# Autodesk Inventor assembly: Clamp with Piston Assembly arpan style
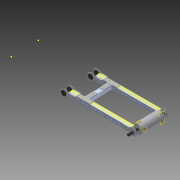
[picture p0: Inventor's stored thumbnail of the model, 180x180]
Saved by Autodesk Inventor 2014 SP1 (Build 180222100, 222)
## iProperties
Created: 2014-01-12
Part Number: Clamp with Piston Assembly arpan style
Document SubType Name: Assembly
Designer: Michael
Mass: 675.185 g
Surface Area: 3066.09 cm^2
Volume: 214.677 cm^3
Density: 3.14511 g/cm^3
Author: Michael
## Documents named in this file (12)
- C:\Users\Arpan\Documents\GitHub\2014buildCAD\New Collector\Clamp with Piston Assembly arpan style.iam
- C:\Users\Arpan\Documents\GitHub\2014buildCAD\New Collector\Vex Pro 1x1 rectangular tubing 14 in length.ipt
- C:\Users\Arpan\Documents\GitHub\2014buildCAD\New Collector\Vex Pro End Bearing Mount.ipt
- C:\Users\Arpan\Documents\GitHub\2014buildCAD\New Collector\Bearing Mount Spacer 1-8 in.ipt
- C:\Users\Arpan\Documents\GitHub\2014buildCAD\New Collector\Vex Pro 1x1 rectangular tubing 6 in length.ipt
- C:\Users\Arpan\Documents\GitHub\2014buildCAD\New Collector\Hex Bearing 3-8 in (FR6ZZL-hex (am-0692)).ipt
- C:\Users\Arpan\Documents\GitHub\2014buildCAD\New Shooter\Vex Pro T gusset.ipt
- C:\Users\Arpan\Documents\GitHub\2014buildCAD\New Shooter\Vex Pro End Bearing Mount.ipt
- C:\Users\Arpan\Documents\GitHub\2014buildCAD\New Shooter\Bearing ID 0.500 Hex OD 1.125.ipt
- C:\Users\Arpan\Documents\GitHub\2014buildCAD\sling shooter\Hex Shaft 1-2 in (am-0856).ipt
- C:\Users\Arpan\Documents\GitHub\2014buildCAD\sling shooter\roller.ipt
- C:\Users\Arpan\Documents\GitHub\2014buildCAD\sling shooter\insert.ipt
## Components (31 placed, 10 different names)
1. Vex Pro 1x1 rectangular tubing 14 in length:1 — Mate:128, Mate:129, Mate:130, Mate:131, Mate:132, Mate:133, Flush:1, Mate:173, Mate:174, Mate:176, Mate:177, Mate:180, Flush:4, Mate:186, Mate:190, Mate:191
2. Vex Pro 1x1 rectangular tubing 14 in length:2 — Mate:150, Mate:151, Mate:152, Mate:153, Mate:154, Mate:155, Mate:172, Flush:2, Flush:3, Mate:182, Mate:187, Mate:188, Mate:189, Mate:196, Mate:197, Mate:205
3. Vex Pro End Bearing Mount:3 — Mate:88, Mate:89, Mate:90, Mate:162, Mate:163
4. Vex Pro End Bearing Mount:4 — Mate:85, Mate:86, Mate:87, Mate:160, Mate:161
5. Bearing Mount Spacer 1-8 in:1 — Mate:85, Mate:86, Mate:87, Mate:125, Mate:126, Mate:127
6. Bearing Mount Spacer 1-8 in:2 — Mate:88, Mate:89, Mate:90, Mate:122, Mate:123, Mate:124
7. Vex Pro 1x1 rectangular tubing 6 in length:2 — Flush:1, Mate:172, Mate:173, Mate:175, Mate:178, Flush:3, Mate:179, Mate:181, Mate:198
8. Bearing Mount Spacer 1-8 in:5 — Mate:122, Mate:123, Mate:124, Mate:128, Mate:129, Mate:130
9. Bearing Mount Spacer 1-8 in:6 — Mate:125, Mate:126, Mate:127, Mate:131, Mate:132, Mate:133
10. Vex Pro End Bearing Mount:5 — Mate:158, Mate:159
11. Bearing Mount Spacer 1-8 in:7
12. Bearing Mount Spacer 1-8 in:8 — Mate:153, Mate:154, Mate:155
13. Vex Pro End Bearing Mount:6 — Mate:156, Mate:157
14. Bearing Mount Spacer 1-8 in:9
15. Bearing Mount Spacer 1-8 in:10 — Mate:150, Mate:151, Mate:152
16. Hex Bearing 3-8 in (FR6ZZL-hex (am-0692)):1 — Mate:160, Mate:161
17. Hex Bearing 3-8 in (FR6ZZL-hex (am-0692)):2 — Mate:162, Mate:163
18. Hex Bearing 3-8 in (FR6ZZL-hex (am-0692)):3 — Mate:156, Mate:157
19. Hex Bearing 3-8 in (FR6ZZL-hex (am-0692)):4 — Mate:158, Mate:159
20. Vex Pro T gusset:1 — Mate:178, Flush:2, Mate:179
21. Vex Pro T gusset:2 — Mate:174, Mate:175, Mate:176, Mate:177
22. Vex Pro T gusset:3 — Mate:180, Flush:4, Mate:181
23. Vex Pro T gusset:4 — Mate:182, Mate:196, Mate:197, Mate:198
24. Vex Pro End Bearing Mount:7 — Mate:186, Mate:190, Mate:191, Mate:192, Mate:193
25. Vex Pro End Bearing Mount:8 — Mate:187, Mate:188, Mate:189, Mate:194, Mate:195
26. Bearing ID 0.500 Hex OD 1.125:1 — Mate:192, Mate:193, Mate:199, Mate:200
27. Bearing ID 0.500 Hex OD 1.125:2 — Mate:194, Mate:195, Flush:5
28. Hex Shaft 1-2 in (am-0856):1 — Mate:199, Mate:200, Flush:5, Mate:203, Mate:204
29. roller:1 — Mate:201, Mate:202, Flush:6, Flush:7
30. insert:1 — Mate:201, Flush:7, Mate:203, Mate:204
31. insert:2 — Mate:202, Flush:6, Mate:205
## Relationships (82: Mate 75, Flush 7)
- Mate:85: Vex Pro End Bearing Mount:4 ↔ Bearing Mount Spacer 1-8 in:1
- Mate:86: Vex Pro End Bearing Mount:4 ↔ Bearing Mount Spacer 1-8 in:1
- Mate:87: Vex Pro End Bearing Mount:4 ↔ Bearing Mount Spacer 1-8 in:1
- Mate:88: Vex Pro End Bearing Mount:3 ↔ Bearing Mount Spacer 1-8 in:2
- Mate:89: Vex Pro End Bearing Mount:3 ↔ Bearing Mount Spacer 1-8 in:2
- Mate:90: Vex Pro End Bearing Mount:3 ↔ Bearing Mount Spacer 1-8 in:2
- Mate:122: Bearing Mount Spacer 1-8 in:2 ↔ Bearing Mount Spacer 1-8 in:5
- Mate:123: Bearing Mount Spacer 1-8 in:2 ↔ Bearing Mount Spacer 1-8 in:5
- Mate:124: Bearing Mount Spacer 1-8 in:2 ↔ Bearing Mount Spacer 1-8 in:5
- Mate:125: Bearing Mount Spacer 1-8 in:1 ↔ Bearing Mount Spacer 1-8 in:6
- Mate:126: Bearing Mount Spacer 1-8 in:1 ↔ Bearing Mount Spacer 1-8 in:6
- Mate:127: Bearing Mount Spacer 1-8 in:1 ↔ Bearing Mount Spacer 1-8 in:6
- Mate:128: Vex Pro 1x1 rectangular tubing 14 in length:1 ↔ Bearing Mount Spacer 1-8 in:5
- Mate:129: Vex Pro 1x1 rectangular tubing 14 in length:1 ↔ Bearing Mount Spacer 1-8 in:5
- Mate:130: Vex Pro 1x1 rectangular tubing 14 in length:1 ↔ Bearing Mount Spacer 1-8 in:5
- Mate:131: Vex Pro 1x1 rectangular tubing 14 in length:1 ↔ Bearing Mount Spacer 1-8 in:6
- Mate:132: Vex Pro 1x1 rectangular tubing 14 in length:1 ↔ Bearing Mount Spacer 1-8 in:6
- Mate:133: Vex Pro 1x1 rectangular tubing 14 in length:1 ↔ Bearing Mount Spacer 1-8 in:6
- [Mate]: Vex Pro End Bearing Mount:5 ↔ Bearing Mount Spacer 1-8 in:7
- [Mate]: Vex Pro End Bearing Mount:5 ↔ Bearing Mount Spacer 1-8 in:7
- [Mate]: Vex Pro End Bearing Mount:5 ↔ Bearing Mount Spacer 1-8 in:7
- [Mate]: Bearing Mount Spacer 1-8 in:7 ↔ Bearing Mount Spacer 1-8 in:8
- [Mate]: Bearing Mount Spacer 1-8 in:7 ↔ Bearing Mount Spacer 1-8 in:8
- [Mate]: Bearing Mount Spacer 1-8 in:7 ↔ Bearing Mount Spacer 1-8 in:8
- [Mate]: Vex Pro End Bearing Mount:6 ↔ Bearing Mount Spacer 1-8 in:9
- [Mate]: Vex Pro End Bearing Mount:6 ↔ Bearing Mount Spacer 1-8 in:9
- [Mate]: Vex Pro End Bearing Mount:6 ↔ Bearing Mount Spacer 1-8 in:9
- [Mate]: Bearing Mount Spacer 1-8 in:9 ↔ Bearing Mount Spacer 1-8 in:10
- [Mate]: Bearing Mount Spacer 1-8 in:9 ↔ Bearing Mount Spacer 1-8 in:10
- [Mate]: Bearing Mount Spacer 1-8 in:9 ↔ Bearing Mount Spacer 1-8 in:10
- Mate:150: Vex Pro 1x1 rectangular tubing 14 in length:2 ↔ Bearing Mount Spacer 1-8 in:10
- Mate:151: Vex Pro 1x1 rectangular tubing 14 in length:2 ↔ Bearing Mount Spacer 1-8 in:10
- Mate:152: Vex Pro 1x1 rectangular tubing 14 in length:2 ↔ Bearing Mount Spacer 1-8 in:10
- Mate:153: Vex Pro 1x1 rectangular tubing 14 in length:2 ↔ Bearing Mount Spacer 1-8 in:8
- Mate:154: Vex Pro 1x1 rectangular tubing 14 in length:2 ↔ Bearing Mount Spacer 1-8 in:8
- Mate:155: Vex Pro 1x1 rectangular tubing 14 in length:2 ↔ Bearing Mount Spacer 1-8 in:8
- Mate:156: Vex Pro End Bearing Mount:6 ↔ Hex Bearing 3-8 in (FR6ZZL-hex (am-0692)):3
- Mate:157: Vex Pro End Bearing Mount:6 ↔ Hex Bearing 3-8 in (FR6ZZL-hex (am-0692)):3
- Mate:158: Vex Pro End Bearing Mount:5 ↔ Hex Bearing 3-8 in (FR6ZZL-hex (am-0692)):4
- Mate:159: Vex Pro End Bearing Mount:5 ↔ Hex Bearing 3-8 in (FR6ZZL-hex (am-0692)):4
- Mate:160: Vex Pro End Bearing Mount:4 ↔ Hex Bearing 3-8 in (FR6ZZL-hex (am-0692)):1
- Mate:161: Vex Pro End Bearing Mount:4 ↔ Hex Bearing 3-8 in (FR6ZZL-hex (am-0692)):1
- Mate:162: Vex Pro End Bearing Mount:3 ↔ Hex Bearing 3-8 in (FR6ZZL-hex (am-0692)):2
- Mate:163: Vex Pro End Bearing Mount:3 ↔ Hex Bearing 3-8 in (FR6ZZL-hex (am-0692)):2
- Flush:1: Vex Pro 1x1 rectangular tubing 14 in length:1 ↔ Vex Pro 1x1 rectangular tubing 6 in length:2
- Mate:172: Vex Pro 1x1 rectangular tubing 14 in length:2 ↔ Vex Pro 1x1 rectangular tubing 6 in length:2
- Mate:173: Vex Pro 1x1 rectangular tubing 14 in length:1 ↔ Vex Pro 1x1 rectangular tubing 6 in length:2
- Mate:174: Vex Pro 1x1 rectangular tubing 14 in length:1 ↔ Vex Pro T gusset:2
- Mate:175: Vex Pro 1x1 rectangular tubing 6 in length:2 ↔ Vex Pro T gusset:2
- Mate:176: Vex Pro 1x1 rectangular tubing 14 in length:1 ↔ Vex Pro T gusset:2
- Mate:177: Vex Pro 1x1 rectangular tubing 14 in length:1 ↔ Vex Pro T gusset:2
- Mate:178: Vex Pro 1x1 rectangular tubing 6 in length:2 ↔ Vex Pro T gusset:1
- Flush:2: Vex Pro 1x1 rectangular tubing 14 in length:2 ↔ Vex Pro T gusset:1
- Flush:3: Vex Pro 1x1 rectangular tubing 14 in length:2 ↔ Vex Pro 1x1 rectangular tubing 6 in length:2
- Mate:179: Vex Pro 1x1 rectangular tubing 6 in length:2 ↔ Vex Pro T gusset:1
- Mate:180: Vex Pro 1x1 rectangular tubing 14 in length:1 ↔ Vex Pro T gusset:3
- Flush:4: Vex Pro 1x1 rectangular tubing 14 in length:1 ↔ Vex Pro T gusset:3
- Mate:181: Vex Pro 1x1 rectangular tubing 6 in length:2 ↔ Vex Pro T gusset:3
- Mate:182: Vex Pro 1x1 rectangular tubing 14 in length:2 ↔ Vex Pro T gusset:4
- Mate:186: Vex Pro 1x1 rectangular tubing 14 in length:1 ↔ Vex Pro End Bearing Mount:7
- Mate:187: Vex Pro 1x1 rectangular tubing 14 in length:2 ↔ Vex Pro End Bearing Mount:8
- Mate:188: Vex Pro 1x1 rectangular tubing 14 in length:2 ↔ Vex Pro End Bearing Mount:8
- Mate:189: Vex Pro 1x1 rectangular tubing 14 in length:2 ↔ Vex Pro End Bearing Mount:8
- Mate:190: Vex Pro 1x1 rectangular tubing 14 in length:1 ↔ Vex Pro End Bearing Mount:7
- Mate:191: Vex Pro 1x1 rectangular tubing 14 in length:1 ↔ Vex Pro End Bearing Mount:7
- Mate:192: Vex Pro End Bearing Mount:7 ↔ Bearing ID 0.500 Hex OD 1.125:1
- Mate:193: Vex Pro End Bearing Mount:7 ↔ Bearing ID 0.500 Hex OD 1.125:1
- Mate:194: Vex Pro End Bearing Mount:8 ↔ Bearing ID 0.500 Hex OD 1.125:2
- Mate:195: Vex Pro End Bearing Mount:8 ↔ Bearing ID 0.500 Hex OD 1.125:2
- Mate:196: Vex Pro 1x1 rectangular tubing 14 in length:2 ↔ Vex Pro T gusset:4
- Mate:197: Vex Pro 1x1 rectangular tubing 14 in length:2 ↔ Vex Pro T gusset:4
- Mate:198: Vex Pro 1x1 rectangular tubing 6 in length:2 ↔ Vex Pro T gusset:4
- Mate:199: Bearing ID 0.500 Hex OD 1.125:1 ↔ Hex Shaft 1-2 in (am-0856):1
- Mate:200: Bearing ID 0.500 Hex OD 1.125:1 ↔ Hex Shaft 1-2 in (am-0856):1
- Flush:5 (11.1125 mm): Bearing ID 0.500 Hex OD 1.125:2 ↔ Hex Shaft 1-2 in (am-0856):1
- Mate:201: roller:1 ↔ insert:1
- Mate:202: roller:1 ↔ insert:2
- Flush:6: roller:1 ↔ insert:2
- Flush:7: roller:1 ↔ insert:1
- Mate:203: Hex Shaft 1-2 in (am-0856):1 ↔ insert:1
- Mate:204: Hex Shaft 1-2 in (am-0856):1 ↔ insert:1
- Mate:205 (3.175 mm): Vex Pro 1x1 rectangular tubing 14 in length:2 ↔ insert:2
## Named parameters: d167_d158 = 0 mm, d168_d159 = 0 mm, d169_d160 = 0 mm, d172_d118 = 0 mm, d173_d119 = 0 mm, d174_d120 = 0 mm, d175_d158 = 0 mm, d176_d159 = 0 mm, d177_d160 = 0 mm, d180_d118 = 0 mm, d181_d119 = 0 mm, d182_d120 = 0 mm
